# Autodesk Inventor assembly: HookHolderAssembly
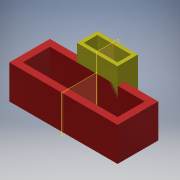
[picture p0: Inventor's stored thumbnail of the model, 180x180]
Saved by Autodesk Inventor 2018.2 (Build 222227000, 227)
## iProperties
Created: 2018-03-20
Part Number: HookHolderAssembly
Document SubType Name: Assembly
Designer: steele
Author: steele
## Documents named in this file (3)
- D:\snobotics\CAD-Development\robSteele\2018-FRC\Hook\HookHolderAssembly.iam
- D:\snobotics\CAD-Development\robSteele\2018-FRC\Hook\magnetHolder.ipt
- D:\snobotics\CAD-Development\robSteele\2018-FRC\Hook\hookSupport.ipt
## Components (2 placed, 2 different names)
1. magnetHolder:1 — Flush:1, Flush:2, Flush:3
2. hookSupport:1 — Flush:1, Flush:2, Flush:3
## Relationships (3: Flush 3)
- Flush:1: magnetHolder:1 ↔ hookSupport:1
- Flush:2: magnetHolder:1 ↔ hookSupport:1
- Flush:3: magnetHolder:1 ↔ hookSupport:1
